# Autodesk Inventor assembly: HitSense
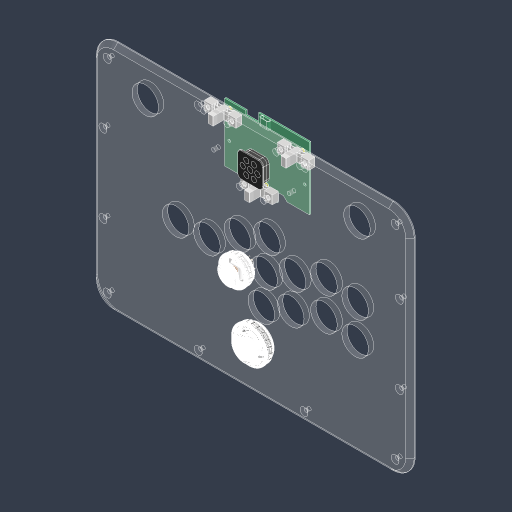
[picture p0: Inventor's stored thumbnail of the model, 512x512]
Saved by Autodesk Inventor 2023.4 (Build 274418000, 418)
## iProperties
Created: 2024-02-20
Part Number: HitSense
Document SubType Name: Assembly
Designer: JoaoSilva
Author: JoaoSilva
## Documents named in this file (17)
- C:\Users\joaos\Documents\GitHub\HitSense\CAD\HitSense.iam
- C:\Users\joaos\Documents\GitHub\HitSense\CAD\30mm_button_cap.ipt
- C:\Users\joaos\Documents\GitHub\HitSense\CAD\30mm_button_nut.ipt
- C:\Users\joaos\Documents\GitHub\HitSense\CAD\24mm_button_body.ipt
- C:\Users\joaos\Documents\GitHub\HitSense\CAD\24mm_button_cap.ipt
- C:\Users\joaos\Documents\GitHub\HitSense\CAD\24mm_button_nut.ipt
- C:\Users\joaos\Documents\GitHub\HitSense\CAD\30mm_button_body.ipt
- C:\Users\joaos\Documents\GitHub\HitSense\CAD\MX_CAD.ipt
- C:\Users\joaos\Documents\GitHub\HitSense\CAD\Top Plate Sanwa.ipt
- C:\Users\joaos\Documents\GitHub\HitSense\CAD\BDM-030.ipt
- C:\Users\joaos\Documents\GitHub\HitSense\CAD\Corner.ipt
- C:\Users\joaos\Documents\GitHub\HitSense\CAD\Corner_MIR.ipt
- C:\Users\joaos\Documents\GitHub\HitSense\CAD\Corner Top Right.ipt
- C:\Users\joaos\Documents\GitHub\HitSense\CAD\Corner Top Left.ipt
- C:\Users\joaos\Documents\GitHub\HitSense\CAD\Bottom Plate Sanwa.ipt
- C:\Users\joaos\Documents\GitHub\HitSense\CAD\Speaker Cover.ipt
- C:\Users\joaos\Documents\GitHub\HitSense\CAD\Actuator.ipt
## Components (19 placed, 16 different names)
1. Top Plate Sanwa:1 — Insert:3, Insert:4, Flush:1, Flush:2, Flush:3, Flush:4, Mate:11, Mate:15, Flush:6, Flush:7, Mate:16, Flush:8, Flush:9, Mate:17, Flush:10, Flush:11, Mate:18, Flush:12, Flush:13, Mate:20, Mate:21, Mate:22, Mate:23, Mate:24, Mate:25
2. Bottom Plate Sanwa:1 — Flush:3, Flush:4, Mate:19
3. BDM-030:1 — Flush:1, Flush:2, Mate:11
4. 30mm_button_cap:1 — Mate:4, Mate:5
5. 30mm_button_nut:1 — Insert:1
6. 30mm_button_body:1 — Insert:1, Mate:1, Mate:2, Mate:3, Insert:3
7. MX_CAD:1 — Mate:1, Mate:2, Mate:3, Mate:4, Mate:5
8. 24mm_button_body:1 — Mate:6, Mate:7, Mate:8, Insert:2, Insert:4
9. 24mm_button_cap:1 — Mate:9, Mate:10
10. 24mm_button_nut:1 — Insert:2
11. MX_CAD:2 — Mate:6, Mate:7, Mate:8, Mate:9, Mate:10
12. Corner:1 — Mate:15, Flush:6, Flush:7, Mate:19
13. Corner_MIR:1 — Mate:16, Flush:8, Flush:9
14. Corner Top Right:1 — Mate:17, Flush:10, Flush:11
15. Corner Top Left:1 — Mate:18, Flush:12, Flush:13
16. Speaker Cover:1 — Mate:20, Mate:21, Mate:22
17. Actuator:1 — Mate:23
18. Actuator:2 — Mate:24
19. Actuator:3 — Mate:25
## Relationships (38: Mate 22, Flush 12, Insert 4)
- Insert:1: 30mm_button_nut:1 ↔ 30mm_button_body:1
- Mate:1: 30mm_button_body:1 ↔ MX_CAD:1
- Mate:2: 30mm_button_body:1 ↔ MX_CAD:1
- Mate:3: 30mm_button_body:1 ↔ MX_CAD:1
- Mate:4: 30mm_button_cap:1 ↔ MX_CAD:1
- Mate:5: 30mm_button_cap:1 ↔ MX_CAD:1
- Mate:6: 24mm_button_body:1 ↔ MX_CAD:2
- Mate:7: 24mm_button_body:1 ↔ MX_CAD:2
- Mate:8: 24mm_button_body:1 ↔ MX_CAD:2
- Insert:2: 24mm_button_body:1 ↔ 24mm_button_nut:1
- Mate:9: 24mm_button_cap:1 ↔ MX_CAD:2
- Mate:10: 24mm_button_cap:1 ↔ MX_CAD:2
- Insert:3: Top Plate Sanwa:1 ↔ 30mm_button_body:1
- Insert:4: Top Plate Sanwa:1 ↔ 24mm_button_body:1
- Flush:1: Top Plate Sanwa:1 ↔ BDM-030:1
- Flush:2 (2 mm): Top Plate Sanwa:1 ↔ BDM-030:1
- Flush:3: Top Plate Sanwa:1 ↔ Bottom Plate Sanwa:1
- Flush:4: Top Plate Sanwa:1 ↔ Bottom Plate Sanwa:1
- Mate:11 (10 mm): Top Plate Sanwa:1 ↔ BDM-030:1
- Mate:15: Top Plate Sanwa:1 ↔ Corner:1
- Flush:6: Top Plate Sanwa:1 ↔ Corner:1
- Flush:7: Top Plate Sanwa:1 ↔ Corner:1
- Mate:16: Top Plate Sanwa:1 ↔ Corner_MIR:1
- Flush:8: Top Plate Sanwa:1 ↔ Corner_MIR:1
- Flush:9: Top Plate Sanwa:1 ↔ Corner_MIR:1
- Mate:17: Top Plate Sanwa:1 ↔ Corner Top Right:1
- Flush:10: Top Plate Sanwa:1 ↔ Corner Top Right:1
- Flush:11: Top Plate Sanwa:1 ↔ Corner Top Right:1
- Mate:18: Top Plate Sanwa:1 ↔ Corner Top Left:1
- Flush:12: Top Plate Sanwa:1 ↔ Corner Top Left:1
- Flush:13: Top Plate Sanwa:1 ↔ Corner Top Left:1
- Mate:19: Bottom Plate Sanwa:1 ↔ Corner:1
- Mate:20: Top Plate Sanwa:1 ↔ Speaker Cover:1
- Mate:21: Top Plate Sanwa:1 ↔ Speaker Cover:1
- Mate:22: Top Plate Sanwa:1 ↔ Speaker Cover:1
- Mate:23: Top Plate Sanwa:1 ↔ Actuator:1
- Mate:24: Top Plate Sanwa:1 ↔ Actuator:2
- Mate:25: Top Plate Sanwa:1 ↔ Actuator:3
